# Autodesk Inventor assembly: SidePanel_GuideRail
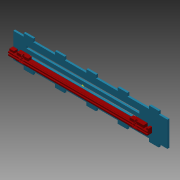
[picture p0: Inventor's stored thumbnail of the model, 180x180]
Saved by Autodesk Inventor 2015 SP1 (Build 190203100, 203)
## iProperties
Created: 2014-08-06
Part Number: SidePanel_GuideRail
Document SubType Name: Assembly
Designer: Patrick Camilleri
Author: Patrick Camilleri
## Documents named in this file (3)
- C:\Users\Patrick Camilleri\CAD\Spin5 Enclosure\SidePanel_GuideRail.iam
- C:\Users\Patrick Camilleri\CAD\Spin5 Enclosure\SidePanel_Rail.ipt
- C:\Users\Patrick Camilleri\CAD\Spin5 Enclosure\GuideRail_24560353.ipt
## Components (2 placed, 2 different names)
1. SidePanel_Rail:1 — Rigid:1
2. GuideRail_24560353:1 — Rigid:1
## Relationships (1: WeldJoint 1)
- Rigid:1 [WeldJoint]: SidePanel_Rail:1 ↔ GuideRail_24560353:1
